# Autodesk Inventor assembly: Assembly1
(part 2 of 8)
610. Coil:316
611. disk holder:159 — Flush:248, Flush:249, Flush:251, Flush:252, Mate:888
612. coin:159
613. Coil:317
614. Coil:318
615. disk holder:160 — Flush:248, Flush:251, Mate:886, Mate:887, Flush:254
616. coin:160
617. Coil:319
618. Coil:320
619. disk holder:161 — Flush:249, Flush:250, Flush:252, Flush:253, Mate:889
620. coin:161
621. Coil:321
622. Coil:322
623. disk holder:162 — Flush:250, Flush:253, Mate:890
624. coin:162
625. Coil:323
626. Coil:324
627. disk holder:163 — Flush:257, Flush:258, Flush:259, Flush:263, Flush:264, Mate:923, Mate:924
628. coin:163
629. Coil:325
630. Coil:326
631. disk holder:164 — Flush:259, Mate:926, Mate:927
632. coin:164
633. Coil:327
634. Coil:328
635. disk holder:165 — Flush:261, Mate:928, Mate:929
636. coin:165
637. Coil:329
638. Coil:330
639. disk holder:166 — Flush:262, Flush:264, Mate:925
640. coin:166
641. Coil:331
642. Coil:332
643. disk holder:167 — Flush:258, Flush:261, Flush:262, Flush:263, Mate:922
644. coin:167
645. Coil:333
646. Coil:334
647. disk holder:168 — Flush:255, Flush:256, Flush:257, Flush:260, Mate:921
648. coin:168
649. Coil:335
650. Coil:336
651. disk holder:169 — Flush:255, Flush:256, Mate:919, Mate:920
652. coin:169
653. Coil:337
654. Coil:338
655. disk holder:170 — Flush:267, Flush:268, Mate:970, Mate:971
656. coin:170
657. Coil:339
658. Coil:340
659. disk holder:171 — Flush:266, Flush:267, Mate:968, Mate:969
660. coin:171
661. Coil:341
662. Coil:342
663. disk holder:172 — Flush:265, Mate:966, Mate:967
664. coin:172
665. Coil:343
666. Coil:344
667. disk holder:173 — Flush:268, Flush:269, Mate:972, Mate:973
668. coin:173
669. Coil:345
670. Coil:346
671. disk holder:174 — Flush:269, Flush:270, Mate:974, Mate:975
672. coin:174
673. Coil:347
674. Coil:348
675. disk holder:175 — Flush:270, Flush:271, Mate:976, Mate:977
676. coin:175
677. Coil:349
678. Coil:350
679. disk holder:176 — Flush:271, Flush:272, Mate:978, Mate:979
680. coin:176
681. Coil:351
682. Coil:352
683. disk holder:177 — Flush:272, Flush:273, Mate:980, Mate:981
684. coin:177
685. Coil:353
686. Coil:354
687. disk holder:178 — Flush:273, Mate:982, Mate:983
688. coin:178
689. Coil:355
690. Coil:356
691. disk holder:179 — Flush:274, Mate:1016, Mate:1017
692. coin:179
693. Coil:357
694. Coil:358
695. disk holder:180 — Flush:277, Flush:280, Mate:1034, Mate:1038
696. coin:180
697. Coil:359
698. Coil:360
699. disk holder:181 — Flush:276, Flush:279, Flush:280, Mate:1035
700. coin:181
701. Coil:361
702. Coil:362
703. disk holder:182 — Flush:275, Flush:276, Flush:278, Flush:279, Mate:1036
704. coin:182
705. Coil:363
706. Coil:364
707. disk holder:183 — Flush:275, Flush:277, Flush:278, Mate:1037
708. coin:183
709. Coil:365
710. Coil:366
## Relationships (1941: Mate 976, Angle 531, Flush 257, RevoluteJoint 177)
- Rotational:1 [RevoluteJoint]: disk holder:1 ↔ coin:1
- Angle:1 (-25 deg): disk holder:1 ↔ coin:1
- Mate:3: disk holder:1 ↔ Coil:1
- Mate:4: disk holder:1 ↔ Coil:1
- Angle:2 (270 deg): disk holder:1 ↔ Coil:1
- Mate:5: disk holder:1 ↔ Coil:2
- Angle:3 (270 deg): disk holder:1 ↔ Coil:2
- Mate:10: disk holder:1 ↔ Coil:2
- Mate:11: FRAME:1
- Mate:12: FRAME:1
- Mate:13: FRAME:1
- Mate:14: disk holder:1
- Mate:15: disk holder:1 ↔ FRAME:1
- Mate:16: disk holder:1 ↔ FRAME:1
- [RevoluteJoint]: disk holder:2 ↔ coin:2
- [Angle] (-25 deg): disk holder:2 ↔ coin:2
- [Mate]: disk holder:2 ↔ Coil:3
- [Mate]: disk holder:2 ↔ Coil:3
- [Angle] (270 deg): disk holder:2 ↔ Coil:3
- [Mate]: disk holder:2 ↔ Coil:4
- [Angle] (270 deg): disk holder:2 ↔ Coil:4
- [Mate]: disk holder:2 ↔ Coil:4
- Mate:21: FRAME:1 ↔ disk holder:2
- Flush:1: FRAME:1 ↔ disk holder:2
- Mate:22: FRAME:1 ↔ disk holder:2
- [RevoluteJoint]: disk holder:3 ↔ coin:3
- [Angle] (-25 deg): disk holder:3 ↔ coin:3
- [Mate]: disk holder:3 ↔ Coil:5
- [Mate]: disk holder:3 ↔ Coil:5
- [Angle] (270 deg): disk holder:3 ↔ Coil:5
- [Mate]: disk holder:3 ↔ Coil:6
- [Angle] (270 deg): disk holder:3 ↔ Coil:6
- [Mate]: disk holder:3 ↔ Coil:6
- Mate:27: FRAME:1 ↔ disk holder:3
- Flush:2: FRAME:1 ↔ disk holder:3
- Mate:28: FRAME:1 ↔ disk holder:3
- [RevoluteJoint]: disk holder:4 ↔ coin:4
- [Angle] (-25 deg): disk holder:4 ↔ coin:4
- [Mate]: disk holder:4 ↔ Coil:7
- [Mate]: disk holder:4 ↔ Coil:7
- [Angle] (270 deg): disk holder:4 ↔ Coil:7
- [Mate]: disk holder:4 ↔ Coil:8
- [Angle] (270 deg): disk holder:4 ↔ Coil:8
- [Mate]: disk holder:4 ↔ Coil:8
- [RevoluteJoint]: disk holder:5 ↔ coin:5
- [Angle] (-25 deg): disk holder:5 ↔ coin:5
- [Mate]: disk holder:5 ↔ Coil:9
- [Mate]: disk holder:5 ↔ Coil:9
- [Angle] (270 deg): disk holder:5 ↔ Coil:9
- [Mate]: disk holder:5 ↔ Coil:10
- [Angle] (270 deg): disk holder:5 ↔ Coil:10
- [Mate]: disk holder:5 ↔ Coil:10
- [RevoluteJoint]: disk holder:6 ↔ coin:6
- [Angle] (-25 deg): disk holder:6 ↔ coin:6
- [Mate]: disk holder:6 ↔ Coil:11
- [Mate]: disk holder:6 ↔ Coil:11
- [Angle] (270 deg): disk holder:6 ↔ Coil:11
- [Mate]: disk holder:6 ↔ Coil:12
- [Angle] (270 deg): disk holder:6 ↔ Coil:12
- [Mate]: disk holder:6 ↔ Coil:12
- [RevoluteJoint]: disk holder:7 ↔ coin:7
- [Angle] (-25 deg): disk holder:7 ↔ coin:7
- [Mate]: disk holder:7 ↔ Coil:13
- [Mate]: disk holder:7 ↔ Coil:13
- [Angle] (270 deg): disk holder:7 ↔ Coil:13
- [Mate]: disk holder:7 ↔ Coil:14
- [Angle] (270 deg): disk holder:7 ↔ Coil:14
- [Mate]: disk holder:7 ↔ Coil:14
- [RevoluteJoint]: disk holder:8 ↔ coin:8
- [Angle] (-25 deg): disk holder:8 ↔ coin:8
- [Mate]: disk holder:8 ↔ Coil:15
- [Mate]: disk holder:8 ↔ Coil:15
- [Angle] (270 deg): disk holder:8 ↔ Coil:15
- [Mate]: disk holder:8 ↔ Coil:16
- [Angle] (270 deg): disk holder:8 ↔ Coil:16
- [Mate]: disk holder:8 ↔ Coil:16
- [RevoluteJoint]: disk holder:9 ↔ coin:9
- [Angle] (-25 deg): disk holder:9 ↔ coin:9
- [Mate]: disk holder:9 ↔ Coil:17
- [Mate]: disk holder:9 ↔ Coil:17
- [Angle] (270 deg): disk holder:9 ↔ Coil:17
- [Mate]: disk holder:9 ↔ Coil:18
- [Angle] (270 deg): disk holder:9 ↔ Coil:18
- [Mate]: disk holder:9 ↔ Coil:18
- [RevoluteJoint]: disk holder:10 ↔ coin:10
- [Angle] (-25 deg): disk holder:10 ↔ coin:10
- [Mate]: disk holder:10 ↔ Coil:19
- [Mate]: disk holder:10 ↔ Coil:19
- [Angle] (270 deg): disk holder:10 ↔ Coil:19
- [Mate]: disk holder:10 ↔ Coil:20
- [Angle] (270 deg): disk holder:10 ↔ Coil:20
- [Mate]: disk holder:10 ↔ Coil:20
- [RevoluteJoint]: disk holder:11 ↔ coin:11
- [Angle] (-25 deg): disk holder:11 ↔ coin:11
- [Mate]: disk holder:11 ↔ Coil:21
- [Mate]: disk holder:11 ↔ Coil:21
- [Angle] (270 deg): disk holder:11 ↔ Coil:21
- [Mate]: disk holder:11 ↔ Coil:22
- [Angle] (270 deg): disk holder:11 ↔ Coil:22
- [Mate]: disk holder:11 ↔ Coil:22
- [RevoluteJoint]: disk holder:12 ↔ coin:12
- [Angle] (-25 deg): disk holder:12 ↔ coin:12
- [Mate]: disk holder:12 ↔ Coil:23
- [Mate]: disk holder:12 ↔ Coil:23
- [Angle] (270 deg): disk holder:12 ↔ Coil:23
- [Mate]: disk holder:12 ↔ Coil:24
- [Angle] (270 deg): disk holder:12 ↔ Coil:24
- [Mate]: disk holder:12 ↔ Coil:24
- [RevoluteJoint]: disk holder:13 ↔ coin:13
- [Angle] (-25 deg): disk holder:13 ↔ coin:13
- [Mate]: disk holder:13 ↔ Coil:25
- [Mate]: disk holder:13 ↔ Coil:25
- [Angle] (270 deg): disk holder:13 ↔ Coil:25
- [Mate]: disk holder:13 ↔ Coil:26
- [Angle] (270 deg): disk holder:13 ↔ Coil:26
- [Mate]: disk holder:13 ↔ Coil:26
- [RevoluteJoint]: disk holder:14 ↔ coin:14
- [Angle] (-25 deg): disk holder:14 ↔ coin:14
- [Mate]: disk holder:14 ↔ Coil:27
- [Mate]: disk holder:14 ↔ Coil:27
- [Angle] (270 deg): disk holder:14 ↔ Coil:27
- [Mate]: disk holder:14 ↔ Coil:28
- [Angle] (270 deg): disk holder:14 ↔ Coil:28
- [Mate]: disk holder:14 ↔ Coil:28
- [RevoluteJoint]: disk holder:15 ↔ coin:15
- [Angle] (-25 deg): disk holder:15 ↔ coin:15
- [Mate]: disk holder:15 ↔ Coil:29
- [Mate]: disk holder:15 ↔ Coil:29
- [Angle] (270 deg): disk holder:15 ↔ Coil:29
- [Mate]: disk holder:15 ↔ Coil:30
- [Angle] (270 deg): disk holder:15 ↔ Coil:30
- [Mate]: disk holder:15 ↔ Coil:30
- Flush:3: FRAME:1 ↔ disk holder:4
- Mate:77: FRAME:1 ↔ disk holder:4
- Mate:78: FRAME:1 ↔ disk holder:4
- Flush:4: FRAME:1 ↔ disk holder:8
- Mate:79: FRAME:1 ↔ disk holder:8
- Mate:80: FRAME:1 ↔ disk holder:8
- Flush:5: FRAME:1 ↔ disk holder:9
- Mate:81: FRAME:1 ↔ disk holder:9
- Mate:82: FRAME:1 ↔ disk holder:9
- Mate:83: FRAME:1 ↔ disk holder:10
- Flush:6: FRAME:1 ↔ disk holder:10
- Mate:84: FRAME:1 ↔ disk holder:10
- Flush:7: FRAME:1 ↔ disk holder:11
- Mate:85: FRAME:1 ↔ disk holder:11
- Mate:86: FRAME:1 ↔ disk holder:11
- Flush:8: FRAME:1 ↔ disk holder:7
- Mate:87: FRAME:1 ↔ disk holder:7
- Mate:88: FRAME:1 ↔ disk holder:7
- Flush:9: FRAME:1 ↔ disk holder:6
- Mate:89: FRAME:1 ↔ disk holder:6
- Mate:90: FRAME:1 ↔ disk holder:6
- Mate:91: FRAME:1 ↔ disk holder:5
- Flush:10: FRAME:1 ↔ disk holder:5
- Mate:92: FRAME:1 ↔ disk holder:5
- Mate:94: FRAME:1 ↔ disk holder:13
- Flush:11: FRAME:1 ↔ disk holder:13
- Mate:95: FRAME:1 ↔ disk holder:12
- Flush:12: FRAME:1 ↔ disk holder:12
- Mate:96: FRAME:1 ↔ disk holder:12
- Flush:13: FRAME:1 ↔ disk holder:15
- Mate:98: FRAME:1 ↔ disk holder:15
- Mate:99: FRAME:1 ↔ disk holder:14
- Flush:14: FRAME:1 ↔ disk holder:14
- Mate:100: FRAME:1 ↔ disk holder:14
- [RevoluteJoint]: disk holder:16 ↔ coin:16
- [Angle] (-25 deg): disk holder:16 ↔ coin:16
- [Mate]: disk holder:16 ↔ Coil:31
- [Mate]: disk holder:16 ↔ Coil:31
- [Angle] (270 deg): disk holder:16 ↔ Coil:31
- [Mate]: disk holder:16 ↔ Coil:32
- [Angle] (270 deg): disk holder:16 ↔ Coil:32
- [Mate]: disk holder:16 ↔ Coil:32
- [RevoluteJoint]: disk holder:17 ↔ coin:17
- [Angle] (-25 deg): disk holder:17 ↔ coin:17
- [Mate]: disk holder:17 ↔ Coil:33
- [Mate]: disk holder:17 ↔ Coil:33
- [Angle] (270 deg): disk holder:17 ↔ Coil:33
- [Mate]: disk holder:17 ↔ Coil:34
- [Angle] (270 deg): disk holder:17 ↔ Coil:34
- [Mate]: disk holder:17 ↔ Coil:34
- [RevoluteJoint]: disk holder:18 ↔ coin:18
- [Angle] (-25 deg): disk holder:18 ↔ coin:18
- [Mate]: disk holder:18 ↔ Coil:35
- [Mate]: disk holder:18 ↔ Coil:35
- [Angle] (270 deg): disk holder:18 ↔ Coil:35
- [Mate]: disk holder:18 ↔ Coil:36
- [Angle] (270 deg): disk holder:18 ↔ Coil:36
- [Mate]: disk holder:18 ↔ Coil:36
- [RevoluteJoint]: disk holder:19 ↔ coin:19
- [Angle] (-25 deg): disk holder:19 ↔ coin:19
- [Mate]: disk holder:19 ↔ Coil:37
- [Mate]: disk holder:19 ↔ Coil:37
- [Angle] (270 deg): disk holder:19 ↔ Coil:37
- [Mate]: disk holder:19 ↔ Coil:38
- [Angle] (270 deg): disk holder:19 ↔ Coil:38
- [Mate]: disk holder:19 ↔ Coil:38
- [RevoluteJoint]: disk holder:20 ↔ coin:20
- [Angle] (-25 deg): disk holder:20 ↔ coin:20
- [Mate]: disk holder:20 ↔ Coil:39
- [Mate]: disk holder:20 ↔ Coil:39
- [Angle] (270 deg): disk holder:20 ↔ Coil:39
- [Mate]: disk holder:20 ↔ Coil:40
- [Angle] (270 deg): disk holder:20 ↔ Coil:40
- [Mate]: disk holder:20 ↔ Coil:40
- Mate:121: FRAME:1 ↔ disk holder:18
- Flush:15: FRAME:1 ↔ disk holder:18
- Mate:122: FRAME:1 ↔ disk holder:18
- Flush:16: FRAME:1 ↔ disk holder:17
- Mate:123: FRAME:1 ↔ disk holder:17
- Mate:124: FRAME:1 ↔ disk holder:17
- Flush:17: FRAME:1 ↔ disk holder:19
- Mate:125: FRAME:1 ↔ disk holder:19
- Mate:126: FRAME:1 ↔ disk holder:19
- Flush:18: FRAME:1 ↔ disk holder:16
- Mate:127: FRAME:1 ↔ disk holder:16
- Mate:128: FRAME:1 ↔ disk holder:16
- Flush:19: FRAME:1 ↔ disk holder:20
- Mate:129: FRAME:1 ↔ disk holder:20
- Mate:130: FRAME:1 ↔ disk holder:20
- [RevoluteJoint]: disk holder:21 ↔ coin:21
- [Angle] (-25 deg): disk holder:21 ↔ coin:21
- [Mate]: disk holder:21 ↔ Coil:41
- [Mate]: disk holder:21 ↔ Coil:41
- [Angle] (270 deg): disk holder:21 ↔ Coil:41
- [Mate]: disk holder:21 ↔ Coil:42
- [Angle] (270 deg): disk holder:21 ↔ Coil:42
- [Mate]: disk holder:21 ↔ Coil:42
- [RevoluteJoint]: disk holder:22 ↔ coin:22
- [Angle] (-25 deg): disk holder:22 ↔ coin:22
- [Mate]: disk holder:22 ↔ Coil:43
- [Mate]: disk holder:22 ↔ Coil:43
- [Angle] (270 deg): disk holder:22 ↔ Coil:43
- [Mate]: disk holder:22 ↔ Coil:44
- [Angle] (270 deg): disk holder:22 ↔ Coil:44
- [Mate]: disk holder:22 ↔ Coil:44
- [RevoluteJoint]: disk holder:23 ↔ coin:23
- [Angle] (-25 deg): disk holder:23 ↔ coin:23
- [Mate]: disk holder:23 ↔ Coil:45
- [Mate]: disk holder:23 ↔ Coil:45
- [Angle] (270 deg): disk holder:23 ↔ Coil:45
- [Mate]: disk holder:23 ↔ Coil:46
- [Angle] (270 deg): disk holder:23 ↔ Coil:46
- [Mate]: disk holder:23 ↔ Coil:46
- [RevoluteJoint]: disk holder:24 ↔ coin:24
- [Angle] (-25 deg): disk holder:24 ↔ coin:24
- [Mate]: disk holder:24 ↔ Coil:47
- [Mate]: disk holder:24 ↔ Coil:47
- [Angle] (270 deg): disk holder:24 ↔ Coil:47
- [Mate]: disk holder:24 ↔ Coil:48
- [Angle] (270 deg): disk holder:24 ↔ Coil:48
- [Mate]: disk holder:24 ↔ Coil:48
- Flush:20: FRAME:1 ↔ disk holder:23
- Mate:147: FRAME:1 ↔ disk holder:23
- Mate:148: FRAME:1 ↔ disk holder:23
- Flush:21: FRAME:1 ↔ disk holder:24
- Mate:149: FRAME:1 ↔ disk holder:24
- Mate:150: FRAME:1 ↔ disk holder:24
- Flush:22: FRAME:1 ↔ disk holder:22
- Mate:151: FRAME:1 ↔ disk holder:22
- Mate:152: FRAME:1 ↔ disk holder:22
- Flush:23: FRAME:1 ↔ disk holder:21
- Mate:153: FRAME:1 ↔ disk holder:21
- Mate:154: FRAME:1 ↔ disk holder:21
- [RevoluteJoint]: disk holder:25 ↔ coin:25
- [Angle] (-25 deg): disk holder:25 ↔ coin:25
- [Mate]: disk holder:25 ↔ Coil:49
- [Mate]: disk holder:25 ↔ Coil:49
- [Angle] (270 deg): disk holder:25 ↔ Coil:49
- [Mate]: disk holder:25 ↔ Coil:50
- [Angle] (270 deg): disk holder:25 ↔ Coil:50
- [Mate]: disk holder:25 ↔ Coil:50
- [RevoluteJoint]: disk holder:26 ↔ coin:26
- [Angle] (-25 deg): disk holder:26 ↔ coin:26
- [Mate]: disk holder:26 ↔ Coil:51
- [Mate]: disk holder:26 ↔ Coil:51
- [Angle] (270 deg): disk holder:26 ↔ Coil:51
- [Mate]: disk holder:26 ↔ Coil:52
- [Angle] (270 deg): disk holder:26 ↔ Coil:52
- [Mate]: disk holder:26 ↔ Coil:52
- [RevoluteJoint]: disk holder:27 ↔ coin:27
- [Angle] (-25 deg): disk holder:27 ↔ coin:27
- [Mate]: disk holder:27 ↔ Coil:53
- [Mate]: disk holder:27 ↔ Coil:53
- [Angle] (270 deg): disk holder:27 ↔ Coil:53
- [Mate]: disk holder:27 ↔ Coil:54
- [Angle] (270 deg): disk holder:27 ↔ Coil:54
- [Mate]: disk holder:27 ↔ Coil:54
- [RevoluteJoint]: disk holder:28 ↔ coin:28
- [Angle] (-25 deg): disk holder:28 ↔ coin:28
- [Mate]: disk holder:28 ↔ Coil:55
- [Mate]: disk holder:28 ↔ Coil:55
- [Angle] (270 deg): disk holder:28 ↔ Coil:55
- [Mate]: disk holder:28 ↔ Coil:56
- [Angle] (270 deg): disk holder:28 ↔ Coil:56
- [Mate]: disk holder:28 ↔ Coil:56
- [RevoluteJoint]: disk holder:29 ↔ coin:29
- [Angle] (-25 deg): disk holder:29 ↔ coin:29
- [Mate]: disk holder:29 ↔ Coil:57
- [Mate]: disk holder:29 ↔ Coil:57
- [Angle] (270 deg): disk holder:29 ↔ Coil:57
- [Mate]: disk holder:29 ↔ Coil:58
- [Angle] (270 deg): disk holder:29 ↔ Coil:58
- [Mate]: disk holder:29 ↔ Coil:58
- [RevoluteJoint]: disk holder:30 ↔ coin:30
- [Angle] (-25 deg): disk holder:30 ↔ coin:30
- [Mate]: disk holder:30 ↔ Coil:59
- [Mate]: disk holder:30 ↔ Coil:59
- [Angle] (270 deg): disk holder:30 ↔ Coil:59
- [Mate]: disk holder:30 ↔ Coil:60
- [Angle] (270 deg): disk holder:30 ↔ Coil:60
- [Mate]: disk holder:30 ↔ Coil:60
- [RevoluteJoint]: disk holder:31 ↔ coin:31
- [Angle] (-25 deg): disk holder:31 ↔ coin:31
- [Mate]: disk holder:31 ↔ Coil:61
- [Mate]: disk holder:31 ↔ Coil:61
- [Angle] (270 deg): disk holder:31 ↔ Coil:61
- [Mate]: disk holder:31 ↔ Coil:62
- [Angle] (270 deg): disk holder:31 ↔ Coil:62
- [Mate]: disk holder:31 ↔ Coil:62
- [RevoluteJoint]: disk holder:32 ↔ coin:32
- [Angle] (-25 deg): disk holder:32 ↔ coin:32
- [Mate]: disk holder:32 ↔ Coil:63
- [Mate]: disk holder:32 ↔ Coil:63
- [Angle] (270 deg): disk holder:32 ↔ Coil:63
- [Mate]: disk holder:32 ↔ Coil:64
- [Angle] (270 deg): disk holder:32 ↔ Coil:64
- [Mate]: disk holder:32 ↔ Coil:64
- [RevoluteJoint]: disk holder:33 ↔ coin:33
- [Angle] (-25 deg): disk holder:33 ↔ coin:33
- [Mate]: disk holder:33 ↔ Coil:65
- [Mate]: disk holder:33 ↔ Coil:65
- [Angle] (270 deg): disk holder:33 ↔ Coil:65
- [Mate]: disk holder:33 ↔ Coil:66
- [Angle] (270 deg): disk holder:33 ↔ Coil:66
- [Mate]: disk holder:33 ↔ Coil:66
- [RevoluteJoint]: disk holder:34 ↔ coin:34
- [Angle] (-25 deg): disk holder:34 ↔ coin:34
- [Mate]: disk holder:34 ↔ Coil:67
- [Mate]: disk holder:34 ↔ Coil:67
- [Angle] (270 deg): disk holder:34 ↔ Coil:67
- [Mate]: disk holder:34 ↔ Coil:68
- [Angle] (270 deg): disk holder:34 ↔ Coil:68
- [Mate]: disk holder:34 ↔ Coil:68
- [RevoluteJoint]: disk holder:35 ↔ coin:35
- [Angle] (-25 deg): disk holder:35 ↔ coin:35
- [Mate]: disk holder:35 ↔ Coil:69
- [Mate]: disk holder:35 ↔ Coil:69
- [Angle] (270 deg): disk holder:35 ↔ Coil:69
- [Mate]: disk holder:35 ↔ Coil:70
- [Angle] (270 deg): disk holder:35 ↔ Coil:70
- [Mate]: disk holder:35 ↔ Coil:70
- [RevoluteJoint]: disk holder:36 ↔ coin:36
- [Angle] (-25 deg): disk holder:36 ↔ coin:36
- [Mate]: disk holder:36 ↔ Coil:71
- [Mate]: disk holder:36 ↔ Coil:71
- [Angle] (270 deg): disk holder:36 ↔ Coil:71
- [Mate]: disk holder:36 ↔ Coil:72
- [Angle] (270 deg): disk holder:36 ↔ Coil:72
- [Mate]: disk holder:36 ↔ Coil:72
- [RevoluteJoint]: disk holder:37 ↔ coin:37
- [Angle] (-25 deg): disk holder:37 ↔ coin:37
- [Mate]: disk holder:37 ↔ Coil:73
- [Mate]: disk holder:37 ↔ Coil:73
- [Angle] (270 deg): disk holder:37 ↔ Coil:73
- [Mate]: disk holder:37 ↔ Coil:74
- [Angle] (270 deg): disk holder:37 ↔ Coil:74
- [Mate]: disk holder:37 ↔ Coil:74
- Flush:24: FRAME:1 ↔ disk holder:32
- Mate:207: FRAME:1 ↔ disk holder:32
- Mate:208: FRAME:1 ↔ disk holder:32
- Flush:25: FRAME:1 ↔ disk holder:29
- Mate:209: FRAME:1 ↔ disk holder:29
- Mate:210: FRAME:1 ↔ disk holder:29
- Flush:26: FRAME:1 ↔ disk holder:33
- Mate:211: FRAME:1 ↔ disk holder:33
- Mate:212: FRAME:1 ↔ disk holder:33
- Flush:27: FRAME:1 ↔ disk holder:28
- Mate:213: FRAME:1 ↔ disk holder:28
- Mate:214: FRAME:1 ↔ disk holder:28
- Flush:28: FRAME:1 ↔ disk holder:34
- Mate:215: FRAME:1 ↔ disk holder:34
- Mate:216: FRAME:1 ↔ disk holder:34
- Flush:29: FRAME:1 ↔ disk holder:31
- Mate:217: FRAME:1 ↔ disk holder:31
- Mate:218: FRAME:1 ↔ disk holder:31
- Flush:30: FRAME:1 ↔ disk holder:25
- Mate:219: FRAME:1 ↔ disk holder:25
- Mate:220: FRAME:1 ↔ disk holder:25
- Flush:31: FRAME:1 ↔ disk holder:30
- Flush:32: FRAME:1 ↔ disk holder:27
- Flush:33: FRAME:1 ↔ disk holder:35
- Flush:34: FRAME:1 ↔ disk holder:36
- Flush:35: FRAME:1 ↔ disk holder:26
- Flush:36: FRAME:1 ↔ disk holder:37
- [RevoluteJoint]: disk holder:38 ↔ coin:38
- [Angle] (-25 deg): disk holder:38 ↔ coin:38
- [Mate]: disk holder:38 ↔ Coil:75
- [Mate]: disk holder:38 ↔ Coil:75
- [Angle] (270 deg): disk holder:38 ↔ Coil:75
- [Mate]: disk holder:38 ↔ Coil:76
- [Angle] (270 deg): disk holder:38 ↔ Coil:76
- [Mate]: disk holder:38 ↔ Coil:76
- [RevoluteJoint]: disk holder:39 ↔ coin:39
- [Angle] (-25 deg): disk holder:39 ↔ coin:39
- [Mate]: disk holder:39 ↔ Coil:77
- [Mate]: disk holder:39 ↔ Coil:77
- [Angle] (270 deg): disk holder:39 ↔ Coil:77
- [Mate]: disk holder:39 ↔ Coil:78
- [Angle] (270 deg): disk holder:39 ↔ Coil:78
- [Mate]: disk holder:39 ↔ Coil:78
- [RevoluteJoint]: disk holder:40 ↔ coin:40
- [Angle] (-25 deg): disk holder:40 ↔ coin:40
- [Mate]: disk holder:40 ↔ Coil:79
- [Mate]: disk holder:40 ↔ Coil:79
- [Angle] (270 deg): disk holder:40 ↔ Coil:79
- [Mate]: disk holder:40 ↔ Coil:80
- [Angle] (270 deg): disk holder:40 ↔ Coil:80
- [Mate]: disk holder:40 ↔ Coil:80
- [RevoluteJoint]: disk holder:41 ↔ coin:41
- [Angle] (-25 deg): disk holder:41 ↔ coin:41
- [Mate]: disk holder:41 ↔ Coil:81
- [Mate]: disk holder:41 ↔ Coil:81
- [Angle] (270 deg): disk holder:41 ↔ Coil:81
- [Mate]: disk holder:41 ↔ Coil:82
- [Angle] (270 deg): disk holder:41 ↔ Coil:82
- [Mate]: disk holder:41 ↔ Coil:82
- [RevoluteJoint]: disk holder:42 ↔ coin:42
- [Angle] (-25 deg): disk holder:42 ↔ coin:42
- [Mate]: disk holder:42 ↔ Coil:83
- [Mate]: disk holder:42 ↔ Coil:83
- [Angle] (270 deg): disk holder:42 ↔ Coil:83
- [Mate]: disk holder:42 ↔ Coil:84
- [Angle] (270 deg): disk holder:42 ↔ Coil:84
- [Mate]: disk holder:42 ↔ Coil:84
- [RevoluteJoint]: disk holder:43 ↔ coin:43
- [Angle] (-25 deg): disk holder:43 ↔ coin:43